# Autodesk Inventor assembly: mppcInterface
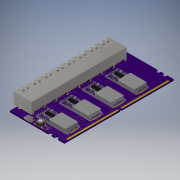
[picture p0: Inventor's stored thumbnail of the model, 180x180]
Saved by Autodesk Inventor 2016 (Build 200138000, 138)
## iProperties
Created: 2016-04-06
Part Number: mppcInterface
Document SubType Name: Assembly
Designer: sawai
Author: sawai
## Documents named in this file (17)
- C:\Users\Jonathan\Documents\Projects\mppcInterface\mppcInterface\cad\mppcInterface.iam
- C:\Users\Jonathan\Documents\Projects\mppcInterface\mppcInterface\cad\mppcInterfacePcb.ipt
- C:\Users\Jonathan\Documents\Projects\mppcInterface\mppcInterface\cad\dependency\mppcHighVoltage\cad\highVoltageMppcBoard.iam
- C:\Users\Jonathan\Documents\Projects\mppcInterface\mppcInterface\cad\connector\SS-668808S-A-PG4-AC.ipt
- C:\Users\Jonathan\Documents\Projects\mppcInterface\mppcInterface\cad\electronics\32 TQFP.ipt
- C:\Users\Jonathan\Documents\Projects\mppcInterface\mppcInterface\cad\electronics\403C.ipt
- C:\Users\Jonathan\Documents\Projects\mppcInterface\mppcInterface\cad\electronics\DX4R005H91.ipt
- C:\Users\Jonathan\Documents\Projects\mppcInterface\mppcInterface\cad\electronics\FSM2JSMAA.ipt
- C:\Users\Jonathan\Documents\Projects\mppcInterface\mppcInterface\cad\electronics\VQFN.ipt
- C:\Users\Jonathan\Documents\Projects\mppcInterface\mppcInterface\cad\electronics\QFN-28.ipt
- C:\Users\Jonathan\Documents\Projects\mppcInterface\mppcInterface\cad\electronics\LXDC2HN18A-097.ipt
- C:\Users\Jonathan\Documents\Projects\mppcInterface\mppcInterface\cad\electronics\soic-8-N.ipt
- C:\Users\Jonathan\Documents\Projects\anodePiShield\coincidenceCounter\cad\electronics\soic\soic.ipt
- C:\Users\Jonathan\Documents\Projects\mppcInterface\mppcInterface\cad\electronics\chipResistor\chipResistor-0402.ipt
- C:\Users\Jonathan\Documents\Projects\dynodePiShield\coincidenceCounter\cad\electronics\resistor\chipResistor.ipt
- C:\Users\Jonathan\Documents\Projects\mppcInterface\mppcInterface\cad\electronics\capacitor\capacitor-0402.ipt
- C:\Users\Jonathan\Documents\Projects\mppcInterface\mppcInterface\cad\electronics\capacitor\capacitor.ipt
## Components (24 placed, 13 different names)
1. mppcInterfacePcb:1 — Angle:1, Angle:2, Mate:1, Mate:2, Angle:3, Mate:3, Mate:4, Angle:4, Mate:5, Mate:7, Angle:6, Mate:8, Mate:9, Mate:10, Mate:11, Angle:8, Mate:12, Angle:9, Mate:13, Angle:10, Mate:14, Angle:11, Angle:12
2. SS-668808S-A-PG4-AC:1 — Angle:2, Mate:3, Angle:7
3. 32 TQFP:1 — Mate:4, Angle:4
4. 403C:1 — Mate:5
5. DX4R005H91:1 — Mate:7, Angle:6
6. FSM2JSMAA:1 — Mate:8
7. VQFN:1 — Mate:9, Angle:7
8. QFN-28:1 — Mate:10
9. LXDC2HN18A-097:1 — Mate:11, Angle:8
10. soic-8-N:1 — Mate:12, Angle:9
11. chipResistor-0402:1 — Mate:13, Angle:10
12. capacitor-0402:1 — Flush:1, Mate:14, Angle:12
13. capacitor-0402:2 — Flush:1, Flush:2
14. capacitor-0402:3 — Flush:2, Flush:3, Flush:4
15. capacitor-0402:4 — Flush:3
16. capacitor-0402:5 — Flush:4, Angle:11
17. highVoltageMppcBoard:1 [sub-assembly] — Angle:1, Mate:1
18. highVoltageMppcBoard:2 [sub-assembly]
19. highVoltageMppcBoard:3 [sub-assembly]
20. highVoltageMppcBoard:4 [sub-assembly]
21. highVoltageMppcBoard:5 [sub-assembly] — Mate:2, Angle:3
22. highVoltageMppcBoard:6 [sub-assembly]
23. highVoltageMppcBoard:7 [sub-assembly]
24. highVoltageMppcBoard:8 [sub-assembly]
## Component patterns: (4 elements, first: highVoltageMppcBoard:1), (4 elements, first: highVoltageMppcBoard:5)
## Relationships (28: Mate 13, Angle 11, Flush 4)
- Angle:1 (180 deg): mppcInterfacePcb:1 ↔ highVoltageMppcBoard:1
- Angle:2 (0 deg): mppcInterfacePcb:1 ↔ SS-668808S-A-PG4-AC:1
- Mate:1: mppcInterfacePcb:1 ↔ highVoltageMppcBoard:1
- Mate:2: mppcInterfacePcb:1 ↔ highVoltageMppcBoard:5
- Angle:3 (0 deg): mppcInterfacePcb:1 ↔ highVoltageMppcBoard:5
- Mate:3: mppcInterfacePcb:1 ↔ SS-668808S-A-PG4-AC:1
- Mate:4: mppcInterfacePcb:1 ↔ 32 TQFP:1
- Angle:4 (0 deg): mppcInterfacePcb:1 ↔ 32 TQFP:1
- Mate:5: mppcInterfacePcb:1 ↔ 403C:1
- Mate:7: mppcInterfacePcb:1 ↔ DX4R005H91:1
- Angle:6 (0 deg): mppcInterfacePcb:1 ↔ DX4R005H91:1
- Mate:8: mppcInterfacePcb:1 ↔ FSM2JSMAA:1
- Mate:9: mppcInterfacePcb:1 ↔ VQFN:1
- Angle:7 (135 deg): SS-668808S-A-PG4-AC:1 ↔ VQFN:1
- Mate:10: mppcInterfacePcb:1 ↔ QFN-28:1
- Mate:11: mppcInterfacePcb:1 ↔ LXDC2HN18A-097:1
- Angle:8 (180 deg): mppcInterfacePcb:1 ↔ LXDC2HN18A-097:1
- Mate:12: mppcInterfacePcb:1 ↔ soic-8-N:1
- Angle:9 (0 deg): mppcInterfacePcb:1 ↔ soic-8-N:1
- Mate:13: mppcInterfacePcb:1 ↔ chipResistor-0402:1
- Angle:10 (0 deg): mppcInterfacePcb:1 ↔ chipResistor-0402:1
- Flush:1: capacitor-0402:1 ↔ capacitor-0402:2
- Flush:2: capacitor-0402:2 ↔ capacitor-0402:3
- Flush:3: capacitor-0402:3 ↔ capacitor-0402:4
- Mate:14: mppcInterfacePcb:1 ↔ capacitor-0402:1
- Flush:4: capacitor-0402:3 ↔ capacitor-0402:5
- Angle:11 (0 deg): mppcInterfacePcb:1 ↔ capacitor-0402:5
- Angle:12 (0 deg): mppcInterfacePcb:1 ↔ capacitor-0402:1
